# Autodesk Inventor assembly: Хроматографический сортировщик
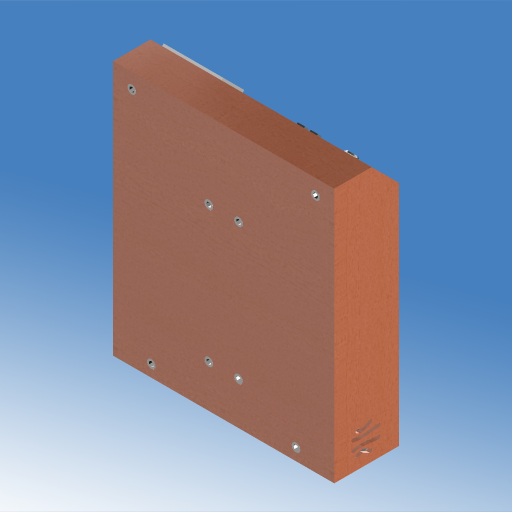
[picture p0: Inventor's stored thumbnail of the model, 512x512]
Saved by Autodesk Inventor 2023 (Build 270158000, 158)
## iProperties
Created: 2022-11-26
Part Number: Хроматографический сортировщик
Document SubType Name: Assembly
Designer: Admin
Author: Admin
## Documents named in this file (32)
- C:\Users\aleks\OneDrive\Рабочий стол\Хроматографический сортировщик\Детали\Хроматографический сортировщик.iam
- C:\Users\aleks\OneDrive\Рабочий стол\Хроматографический сортировщик\Детали\Корпус.ipt
- C:\Users\aleks\OneDrive\Рабочий стол\Хроматографический сортировщик\Детали\Барабан.ipt
- C:\Users\aleks\OneDrive\Рабочий стол\Хроматографический сортировщик\Детали\Короб подшипника.ipt
- C:\Users\aleks\OneDrive\Рабочий стол\Хроматографический сортировщик\Детали\Покупные\Болт М5.ipt
- C:\Users\aleks\OneDrive\Рабочий стол\Хроматографический сортировщик\Детали\Покупные\Гайка М5 стопорная.ipt
- C:\Users\aleks\OneDrive\Рабочий стол\Хроматографический сортировщик\Детали\Покупные\Подшипник.ipt
- C:\Users\aleks\OneDrive\Рабочий стол\Хроматографический сортировщик\Детали\Покупные\Оптический датчик.ipt
- C:\Users\aleks\OneDrive\Рабочий стол\Хроматографический сортировщик\Детали\Покупные\Свая.ipt
- C:\Users\aleks\OneDrive\Рабочий стол\Хроматографический сортировщик\Детали\Покупные\Шаговик\Вал.ipt
- C:\Users\aleks\OneDrive\Рабочий стол\Хроматографический сортировщик\Детали\Покупные\Шаговик\Шаговый мотор.ipt
- C:\Users\aleks\OneDrive\Рабочий стол\Хроматографический сортировщик\Детали\Шевронная маленькая шестерня под мотор.ipt
- C:\Users\aleks\OneDrive\Рабочий стол\Хроматографический сортировщик\Детали\Шевронная планетарная шестерня.ipt
- C:\Users\aleks\OneDrive\Рабочий стол\Хроматографический сортировщик\Детали\Шевронная шестерня для энкодера.ipt
- C:\Users\aleks\OneDrive\Рабочий стол\Хроматографический сортировщик\Детали\Крепёж оптического датчика.ipt
- C:\Users\aleks\OneDrive\Рабочий стол\Хроматографический сортировщик\Детали\Колесо энкодера.ipt
- C:\Users\aleks\OneDrive\Рабочий стол\Хроматографический сортировщик\Детали\Покупные\Болт М3.ipt
- C:\Users\aleks\OneDrive\Рабочий стол\Хроматографический сортировщик\Детали\Покупные\Гайка М3.ipt
- C:\Users\aleks\OneDrive\Рабочий стол\Хроматографический сортировщик\Детали\Покупные\Лазер маленький.ipt
- C:\Users\aleks\OneDrive\Рабочий стол\Хроматографический сортировщик\Детали\Покупные\Лазер.ipt
- C:\Users\aleks\OneDrive\Рабочий стол\Хроматографический сортировщик\Детали\Покупные\Динамик\Динамик.ipt
- C:\Users\aleks\OneDrive\Рабочий стол\Хроматографический сортировщик\Детали\Табличка.ipt
- C:\Users\aleks\OneDrive\Рабочий стол\Хроматографический сортировщик\Детали\Покупные\Кнопки на плате.iam
- C:\Users\aleks\OneDrive\Рабочий стол\Хроматографический сортировщик\Детали\Покупные\Дисплей.ipt
- C:\Users\aleks\OneDrive\Рабочий стол\Хроматографический сортировщик\Детали\Покупные\Кнопка.ipt
- C:\Users\aleks\OneDrive\Рабочий стол\Хроматографический сортировщик\Детали\Колбы\Модель колба коническая 50мл.ipt
- C:\Users\aleks\OneDrive\Рабочий стол\Хроматографический сортировщик\Детали\Покупные\Плата главная.ipt
- C:\Users\aleks\OneDrive\Рабочий стол\Хроматографический сортировщик\Детали\Покупные\Разъём питания.ipt
- C:\Users\aleks\OneDrive\Рабочий стол\Хроматографический сортировщик\Детали\Покупные\Болт М6.ipt
- C:\Users\aleks\OneDrive\Рабочий стол\Хроматографический сортировщик\Детали\Покупные\Гайка М6.ipt
- C:\Users\aleks\OneDrive\Рабочий стол\Хроматографический сортировщик\Детали\Покупные\Болт М4.ipt
- C:\Users\aleks\OneDrive\Рабочий стол\Хроматографический сортировщик\Детали\Покупные\Гайка М4.ipt
## Components (99 placed, 31 different names)
1. Корпус:1 — Совмещение:38, Заподлицо:1, Совмещение:39, Совмещение:40, Заподлицо:2, Совмещение:41, Совмещение:42, Совмещение:43, Совмещение:44, Совмещение:51, Совмещение:52, Совмещение:53, Угол:3, Угол:4, Совмещение:72, Совмещение:73, Совмещение:74, Заподлицо:6, Совмещение:75, Совмещение:76, Совмещение:77, Совмещение:78, Совмещение:80, Угол:5, Совмещение:81, Угол:6, Совмещение:82, Совмещение:85, Совмещение:86, Совмещение:87, Совмещение:88, Совмещение:89, Совмещение:91, Совмещение:92, Совмещение:93, Совмещение:94, Совмещение:96, Совмещение:97, Совмещение:98, Совмещение:101, Совмещение:102, Совмещение:103, Совмещение:104, Совмещение:128, Совмещение:129, Совмещение:130, Совмещение:131, Совмещение:132, Совмещение:133, Совмещение:134, Совмещение:137, Совмещение:138, Совмещение:139, Совмещение:140, Совмещение:141, Совмещение:142, Заподлицо:17, Заподлицо:18, Заподлицо:19, Заподлицо:20, Заподлицо:21, Заподлицо:22, Заподлицо:23, Заподлицо:24, Угол:7, Угол:8, Угол:9, Угол:10, Совмещение:148, Угол:11, Заподлицо:27, Угол:12, Угол:13, Заподлицо:28, Совмещение:156, Совмещение:157, Совмещение:158, Совмещение:159, Угол:15, Угол:16, Угол:17, Угол:18, Заподлицо:29, Заподлицо:30, Заподлицо:31, Заподлицо:32, Совмещение:164, Совмещение:165, Совмещение:166, Совмещение:167, Совмещение:168, Совмещение:169, Совмещение:170, Совмещение:171, Совмещение:172, Угол:19, Угол:20, Угол:21, Угол:22, Заподлицо:36, Заподлицо:37, Заподлицо:38, Заподлицо:39, Заподлицо:40, Заподлицо:41, Заподлицо:42, Заподлицо:43, Угол:23, Угол:24, Угол:25, Угол:26
2. Барабан:1 — Совмещение:25, Совмещение:27, Совмещение:28, Совмещение:29, Совмещение:30, Совмещение:31, Совмещение:32, Совмещение:33, Совмещение:34, Совмещение:35, Совмещение:36, Совмещение:37, Совмещение:38, Заподлицо:1, Совмещение:49, ЗубчПер:5, Совмещение:108, Совмещение:109, Совмещение:110, Совмещение:111, Совмещение:112, Совмещение:113, Совмещение:114, Совмещение:115, Совмещение:116, Совмещение:117, Совмещение:118, Совмещение:119, Совмещение:120, Совмещение:121, Совмещение:122, Совмещение:123
3. Короб подшипника:1 — Совмещение:3, Совмещение:13, Совмещение:17, Совмещение:18, Совмещение:25, Совмещение:27, Совмещение:28
4. Короб подшипника:2 — Совмещение:4, Совмещение:10, Совмещение:16, Совмещение:23, Совмещение:24, Совмещение:29, Совмещение:30, Совмещение:31
5. Короб подшипника:3 — Совмещение:1, Совмещение:15, Совмещение:21, Совмещение:22, Совмещение:32, Совмещение:33, Совмещение:34
6. Короб подшипника:4 — Совмещение:2, Совмещение:14, Совмещение:19, Совмещение:20, Совмещение:35, Совмещение:36, Совмещение:37
7. Болт М5:1 — Совмещение:11, Совмещение:20
8. Гайка М5 стопорная:1 — Совмещение:8, Совмещение:19
9. Подшипник:1 — Совмещение:2, Совмещение:8, Совмещение:11, Совмещение:14
10. Болт М5:2 — Совмещение:12, Совмещение:22
11. Гайка М5 стопорная:2 — Совмещение:7, Совмещение:12, Совмещение:21
12. Подшипник:2 — Совмещение:1, Совмещение:7, Совмещение:15
13. Болт М5:3 — Совмещение:10, Совмещение:24
14. Гайка М5 стопорная:3 — Совмещение:6, Совмещение:23
15. Подшипник:3 — Совмещение:4, Совмещение:6, Совмещение:16
16. Болт М5:4 — Совмещение:9, Совмещение:18
17. Гайка М5 стопорная:4 — Совмещение:5, Совмещение:17
18. Подшипник:4 — Совмещение:3, Совмещение:5, Совмещение:9, Совмещение:13
19. Оптический датчик:1 — Совмещение:54, Совмещение:55, Совмещение:56, Совмещение:58, Совмещение:63, Совмещение:64
20. Подшипник:5 — Совмещение:40, Заподлицо:2
21. Свая:1 — Совмещение:39, Совмещение:41, Совмещение:50, Заподлицо:4, Совмещение:57, ЗубчПер:4
22. Вал:1 — Совмещение:45, Совмещение:46, Совмещение:154, Совмещение:155, Угол:14
23. Шаговый мотор:1 — Совмещение:42, Совмещение:43, Совмещение:44, Совмещение:45, Совмещение:46, Совмещение:149, Совмещение:150, Совмещение:151
24. Шевронная маленькая шестерня под мотор:1 — Заподлицо:3, ЗубчПер:1, ЗубчПер:2, Совмещение:154, Совмещение:155, Угол:14
25. Шевронная планетарная шестерня:1 — Совмещение:49, Заподлицо:3, ЗубчПер:2, ЗубчПер:5
26. Шевронная шестерня для энкодера:1 — Совмещение:50, Заподлицо:4, ЗубчПер:1, ЗубчПер:3, ЗубчПер:4
27. Крепёж оптического датчика:1 — Совмещение:51, Совмещение:52, Совмещение:53, Совмещение:54, Совмещение:55, Совмещение:56, Совмещение:59, Совмещение:60, Совмещение:61, Совмещение:62, Совмещение:65, Совмещение:68, Угол:1, Совмещение:69, Угол:2
28. Колесо энкодера:1 — Совмещение:57, Совмещение:58, ЗубчПер:3
29. Болт М3:1 — Совмещение:59, Заподлицо:5, Совмещение:71
30. Болт М3:2 — Совмещение:60, Заподлицо:5, Совмещение:65, Совмещение:70
31. Болт М3:3 — Совмещение:61, Совмещение:63, Совмещение:66, ЗубчПер:6
32. Болт М3:4 — Совмещение:62, Совмещение:64, Совмещение:67, ЗубчПер:7
33. Гайка М3:1 — Совмещение:71, Угол:4, Совмещение:72
34. Гайка М3:2 — Совмещение:70, Угол:3, Совмещение:73
35. Гайка М3:3 — Совмещение:66, Совмещение:68, Угол:1, ЗубчПер:6
36. Гайка М3:4 — Совмещение:67, Совмещение:69, Угол:2, ЗубчПер:7
37. Лазер маленький:1 — Совмещение:75, Совмещение:77
38. Лазер маленький:2 — Совмещение:76, Совмещение:78
39. Лазер:1 — Совмещение:74, Заподлицо:6
40. Болт М3:5 — Совмещение:84, Совмещение:85
41. Болт М3:6 — Совмещение:83, Совмещение:86
42. Гайка М3:5 — Совмещение:80, Угол:5, Заподлицо:7, Совмещение:83
43. Гайка М3:6 — Совмещение:81, Угол:6, Заподлицо:7, Совмещение:82, Совмещение:84
44. Динамик:1 — Совмещение:87, Совмещение:90
45. Динамик:2 — Совмещение:88, Совмещение:89, Совмещение:90
46. Табличка:1 — Совмещение:91, Совмещение:92, Совмещение:93
47. Кнопки на плате:1 [sub-assembly] — Совмещение:97, Совмещение:98, Совмещение:104
48. Дисплей:1 — Совмещение:96, Совмещение:102, Совмещение:103
49. Кнопка:1 — Совмещение:94, Совмещение:101
50. Модель колба коническая 50мл:1 — Совмещение:114, Совмещение:122
51. Модель колба коническая 50мл:2 — Совмещение:115, Совмещение:121
52. Модель колба коническая 50мл:3 — Совмещение:110, Совмещение:118
53. Модель колба коническая 50мл:4 — Совмещение:113, Совмещение:123
54. Модель колба коническая 50мл:5 — Совмещение:112, Совмещение:116
55. Модель колба коническая 50мл:6 — Совмещение:111, Совмещение:117
56. Модель колба коническая 50мл:7 — Совмещение:109, Совмещение:119
57. Модель колба коническая 50мл:8 — Совмещение:108, Совмещение:120
58. Плата главная:1 — Совмещение:124, Совмещение:125, Совмещение:126, Совмещение:127, Совмещение:129, Совмещение:135, Совмещение:136
59. Болт М3:7 — Заподлицо:8, Совмещение:124, Заподлицо:16, Совмещение:179
60. Болт М3:8 — Заподлицо:9, Заподлицо:10, Совмещение:126, Заподлицо:14, Заподлицо:15, Совмещение:177
61. Болт М3:9 — Заподлицо:10, Совмещение:125, Заподлицо:14, Совмещение:178
62. Болт М3:10 — Заподлицо:8, Заподлицо:9, Совмещение:127, Совмещение:128, Заподлицо:15, Заподлицо:16, Совмещение:136, Совмещение:180
63. Гайка М3:7 — Совмещение:133, Совмещение:134, Заподлицо:11
64. Гайка М3:8 — Совмещение:131, Заподлицо:12, Совмещение:135
65. Гайка М3:9 — Совмещение:132, Заподлицо:11, Заподлицо:12, Заподлицо:13
66. Гайка М3:10 — Совмещение:130, Заподлицо:13
67. Разъём питания:1 — Совмещение:137, Совмещение:138
68. Болт М6:1 — Совмещение:141, Заподлицо:17, Совмещение:147
69. Болт М6:2 — Совмещение:140, Заподлицо:20, Совмещение:146
70. Болт М6:3 — Совмещение:142, Заподлицо:18, Совмещение:144
71. Болт М6:4 — Совмещение:139, Заподлицо:19, Совмещение:143
72. Гайка М6:1 — Совмещение:144, Заподлицо:24, Угол:7
73. Гайка М6:2 — Совмещение:143, Заподлицо:23, Угол:8
74. Гайка М6:3 — Совмещение:146, Заподлицо:21, Угол:10
75. Гайка М6:4 — Совмещение:147, Заподлицо:22, Угол:9
76. Болт М4:1 — Совмещение:149, Заподлицо:26, Совмещение:153
77. Гайка М4:1 — Совмещение:152, Угол:13, Заподлицо:28
78. Болт М4:2 — Совмещение:150, Заподлицо:26, Совмещение:151, Совмещение:152
79. Гайка М4:2 — Совмещение:153, Заподлицо:27, Угол:12
80. Болт М3:11 — Совмещение:158, Совмещение:161, Заподлицо:34
81. Гайка М3:11 — Совмещение:162, Угол:16, Заподлицо:29
82. Болт М3:12 — Совмещение:156, Совмещение:162, Заподлицо:34, Заподлицо:35
83. Гайка М3:12 — Совмещение:160, Угол:15, Заподлицо:30
84. Болт М3:13 — Совмещение:157, Совмещение:160, Заподлицо:33, Заподлицо:35, Совмещение:164
85. Гайка М3:13 — Совмещение:161, Угол:17, Заподлицо:31
86. Болт М3:14 — Совмещение:159, Совмещение:163, Заподлицо:33
87. Гайка М3:14 — Совмещение:163, Угол:18, Заподлицо:32
88. Болт М6:5 — Совмещение:168, Совмещение:176, Заподлицо:38
89. Гайка М6:5 — Совмещение:169, Угол:21, Совмещение:176
90. Болт М6:6 — Совмещение:166, Совмещение:173, Заподлицо:37
91. Гайка М6:6 — Совмещение:170, Угол:22, Совмещение:175
92. Болт М6:7 — Совмещение:165, Совмещение:174, Заподлицо:36
93. Гайка М6:7 — Совмещение:172, Угол:19, Совмещение:173
94. Болт М6:8 — Совмещение:167, Совмещение:175, Заподлицо:39
95. Гайка М6:8 — Совмещение:171, Угол:20, Совмещение:174
96. Гайка М3:15 — Совмещение:177, Заподлицо:41, Угол:25
97. Гайка М3:16 — Совмещение:178, Заподлицо:42, Угол:24
98. Гайка М3:17 — Совмещение:179, Заподлицо:43, Угол:23
99. Гайка М3:18 — Совмещение:180, Заподлицо:40, Угол:26
## Relationships (245: Mate 169, Flush 43, Angle 26, RelateRotation 7)
- Совмещение:1 [Mate]: Короб подшипника:3 ↔ Подшипник:2
- Совмещение:2 [Mate]: Короб подшипника:4 ↔ Подшипник:1
- Совмещение:3 [Mate]: Короб подшипника:1 ↔ Подшипник:4
- Совмещение:4 [Mate]: Короб подшипника:2 ↔ Подшипник:3
- Совмещение:5 [Mate]: Гайка М5 стопорная:4 ↔ Подшипник:4
- Совмещение:6 [Mate]: Гайка М5 стопорная:3 ↔ Подшипник:3
- Совмещение:7 [Mate]: Гайка М5 стопорная:2 ↔ Подшипник:2
- Совмещение:8 [Mate]: Гайка М5 стопорная:1 ↔ Подшипник:1
- Совмещение:9 [Mate]: Болт М5:4 ↔ Подшипник:4
- Совмещение:10 [Mate]: Короб подшипника:2 ↔ Болт М5:3
- Совмещение:11 [Mate]: Болт М5:1 ↔ Подшипник:1
- Совмещение:12 [Mate]: Болт М5:2 ↔ Гайка М5 стопорная:2
- Совмещение:13 [Mate] (0.5 mm): Короб подшипника:1 ↔ Подшипник:4
- Совмещение:14 [Mate] (0.5 mm): Короб подшипника:4 ↔ Подшипник:1
- Совмещение:15 [Mate] (0.5 mm): Короб подшипника:3 ↔ Подшипник:2
- Совмещение:16 [Mate] (0.5 mm): Короб подшипника:2 ↔ Подшипник:3
- Совмещение:17 [Mate]: Короб подшипника:1 ↔ Гайка М5 стопорная:4
- Совмещение:18 [Mate]: Короб подшипника:1 ↔ Болт М5:4
- Совмещение:19 [Mate]: Короб подшипника:4 ↔ Гайка М5 стопорная:1
- Совмещение:20 [Mate]: Короб подшипника:4 ↔ Болт М5:1
- Совмещение:21 [Mate]: Короб подшипника:3 ↔ Гайка М5 стопорная:2
- Совмещение:22 [Mate]: Короб подшипника:3 ↔ Болт М5:2
- Совмещение:23 [Mate]: Короб подшипника:2 ↔ Гайка М5 стопорная:3
- Совмещение:24 [Mate]: Короб подшипника:2 ↔ Болт М5:3
- Совмещение:25 [Mate] (0.1 mm): Барабан:1 ↔ Короб подшипника:1
- Совмещение:27 [Mate]: Барабан:1 ↔ Короб подшипника:1
- Совмещение:28 [Mate] (0.1 mm): Барабан:1 ↔ Короб подшипника:1
- Совмещение:29 [Mate] (0.1 mm): Барабан:1 ↔ Короб подшипника:2
- Совмещение:30 [Mate] (0.1 mm): Барабан:1 ↔ Короб подшипника:2
- Совмещение:31 [Mate]: Барабан:1 ↔ Короб подшипника:2
- Совмещение:32 [Mate] (0.1 mm): Барабан:1 ↔ Короб подшипника:3
- Совмещение:33 [Mate] (0.1 mm): Барабан:1 ↔ Короб подшипника:3
- Совмещение:34 [Mate]: Барабан:1 ↔ Короб подшипника:3
- Совмещение:35 [Mate]: Барабан:1 ↔ Короб подшипника:4
- Совмещение:36 [Mate] (0.1 mm): Барабан:1 ↔ Короб подшипника:4
- Совмещение:37 [Mate] (0.1 mm): Барабан:1 ↔ Короб подшипника:4
- Совмещение:38 [Mate]: Корпус:1 ↔ Барабан:1
- Заподлицо:1 [Flush] (-62.5 mm): Корпус:1 ↔ Барабан:1
- Совмещение:39 [Mate]: Корпус:1 ↔ Свая:1
- Совмещение:40 [Mate]: Корпус:1 ↔ Подшипник:5
- Заподлицо:2 [Flush]: Корпус:1 ↔ Подшипник:5
- Совмещение:41 [Mate]: Корпус:1 ↔ Свая:1
- Совмещение:42 [Mate]: Корпус:1 ↔ Шаговый мотор:1
- Совмещение:43 [Mate]: Корпус:1 ↔ Шаговый мотор:1
- Совмещение:44 [Mate]: Корпус:1 ↔ Шаговый мотор:1
- Совмещение:45 [Mate]: Вал:1 ↔ Шаговый мотор:1
- Совмещение:46 [Mate]: Вал:1 ↔ Шаговый мотор:1
- Совмещение:49 [Mate]: Барабан:1 ↔ Шевронная планетарная шестерня:1
- Заподлицо:3 [Flush]: Шевронная маленькая шестерня под мотор:1 ↔ Шевронная планетарная шестерня:1
- Совмещение:50 [Mate]: Свая:1 ↔ Шевронная шестерня для энкодера:1
- Заподлицо:4 [Flush]: Свая:1 ↔ Шевронная шестерня для энкодера:1
- ЗубчПер:1 [RelateRotation] (1 ul): Шевронная маленькая шестерня под мотор:1 ↔ Шевронная шестерня для энкодера:1
- ЗубчПер:2 [RelateRotation] (0.375 ul): Шевронная маленькая шестерня под мотор:1 ↔ Шевронная планетарная шестерня:1
- Совмещение:51 [Mate]: Корпус:1 ↔ Крепёж оптического датчика:1
- Совмещение:52 [Mate]: Корпус:1 ↔ Крепёж оптического датчика:1
- Совмещение:53 [Mate]: Корпус:1 ↔ Крепёж оптического датчика:1
- Совмещение:54 [Mate]: Оптический датчик:1 ↔ Крепёж оптического датчика:1
- Совмещение:55 [Mate]: Оптический датчик:1 ↔ Крепёж оптического датчика:1
- Совмещение:56 [Mate]: Оптический датчик:1 ↔ Крепёж оптического датчика:1
- Совмещение:57 [Mate]: Свая:1 ↔ Колесо энкодера:1
- Совмещение:58 [Mate]: Оптический датчик:1 ↔ Колесо энкодера:1
- ЗубчПер:3 [RelateRotation] (1 ul): Шевронная шестерня для энкодера:1 ↔ Колесо энкодера:1
- ЗубчПер:4 [RelateRotation] (1 ul): Свая:1 ↔ Шевронная шестерня для энкодера:1
- ЗубчПер:5 [RelateRotation] (1 ul): Барабан:1 ↔ Шевронная планетарная шестерня:1
- Совмещение:59 [Mate]: Крепёж оптического датчика:1 ↔ Болт М3:1
- Совмещение:60 [Mate]: Крепёж оптического датчика:1 ↔ Болт М3:2
- Совмещение:61 [Mate]: Крепёж оптического датчика:1 ↔ Болт М3:3
- Совмещение:62 [Mate]: Крепёж оптического датчика:1 ↔ Болт М3:4
- Совмещение:63 [Mate]: Оптический датчик:1 ↔ Болт М3:3
- Совмещение:64 [Mate]: Оптический датчик:1 ↔ Болт М3:4
- Заподлицо:5 [Flush]: Болт М3:1 ↔ Болт М3:2
- Совмещение:65 [Mate]: Крепёж оптического датчика:1 ↔ Болт М3:2
- Совмещение:66 [Mate]: Болт М3:3 ↔ Гайка М3:3
- Совмещение:67 [Mate]: Болт М3:4 ↔ Гайка М3:4
- Совмещение:68 [Mate]: Крепёж оптического датчика:1 ↔ Гайка М3:3
- Угол:1 [Angle] (0 deg): Крепёж оптического датчика:1 ↔ Гайка М3:3
- Совмещение:69 [Mate]: Крепёж оптического датчика:1 ↔ Гайка М3:4
- Угол:2 [Angle] (0 deg): Крепёж оптического датчика:1 ↔ Гайка М3:4
- ЗубчПер:6 [RelateRotation] (1 ul): Болт М3:3 ↔ Гайка М3:3
- ЗубчПер:7 [RelateRotation] (1 ul): Болт М3:4 ↔ Гайка М3:4
- Совмещение:70 [Mate]: Болт М3:2 ↔ Гайка М3:2
- Совмещение:71 [Mate]: Болт М3:1 ↔ Гайка М3:1
- Угол:3 [Angle] (0 deg): Корпус:1 ↔ Гайка М3:2
- Угол:4 [Angle] (0 deg): Корпус:1 ↔ Гайка М3:1
- Совмещение:72 [Mate]: Корпус:1 ↔ Гайка М3:1
- Совмещение:73 [Mate]: Корпус:1 ↔ Гайка М3:2
- Совмещение:74 [Mate]: Корпус:1 ↔ Лазер:1
- Заподлицо:6 [Flush]: Корпус:1 ↔ Лазер:1
- Совмещение:75 [Mate]: Корпус:1 ↔ Лазер маленький:1
- Совмещение:76 [Mate]: Корпус:1 ↔ Лазер маленький:2
- Совмещение:77 [Mate]: Корпус:1 ↔ Лазер маленький:1
- Совмещение:78 [Mate]: Корпус:1 ↔ Лазер маленький:2
- Совмещение:80 [Mate]: Корпус:1 ↔ Гайка М3:5
- Угол:5 [Angle] (0 deg): Корпус:1 ↔ Гайка М3:5
- Совмещение:81 [Mate]: Корпус:1 ↔ Гайка М3:6
- Угол:6 [Angle] (0 deg): Корпус:1 ↔ Гайка М3:6
- Заподлицо:7 [Flush]: Гайка М3:5 ↔ Гайка М3:6
- Совмещение:82 [Mate]: Корпус:1 ↔ Гайка М3:6
- Совмещение:83 [Mate]: Болт М3:6 ↔ Гайка М3:5
- Совмещение:84 [Mate]: Болт М3:5 ↔ Гайка М3:6
- Совмещение:85 [Mate]: Корпус:1 ↔ Болт М3:5
- Совмещение:86 [Mate]: Корпус:1 ↔ Болт М3:6
- Совмещение:87 [Mate]: Корпус:1 ↔ Динамик:1
- Совмещение:88 [Mate]: Корпус:1 ↔ Динамик:2
- Совмещение:89 [Mate]: Корпус:1 ↔ Динамик:2
- Совмещение:90 [Mate]: Динамик:1 ↔ Динамик:2
- Совмещение:91 [Mate]: Корпус:1 ↔ Табличка:1
- Совмещение:92 [Mate]: Корпус:1 ↔ Табличка:1
- Совмещение:93 [Mate]: Корпус:1 ↔ Табличка:1
- Совмещение:94 [Mate]: Корпус:1 ↔ Кнопка:1
- Совмещение:96 [Mate]: Корпус:1 ↔ Дисплей:1
- Совмещение:97 [Mate]: Корпус:1 ↔ Кнопки на плате:1
- Совмещение:98 [Mate]: Корпус:1 ↔ Кнопки на плате:1
- Совмещение:101 [Mate]: Корпус:1 ↔ Кнопка:1
- Совмещение:102 [Mate]: Корпус:1 ↔ Дисплей:1
- Совмещение:103 [Mate]: Корпус:1 ↔ Дисплей:1
- Совмещение:104 [Mate]: Корпус:1 ↔ Кнопки на плате:1
- Совмещение:108 [Mate]: Барабан:1 ↔ Модель колба коническая 50мл:8
- Совмещение:109 [Mate]: Барабан:1 ↔ Модель колба коническая 50мл:7
- Совмещение:110 [Mate]: Барабан:1 ↔ Модель колба коническая 50мл:3
- Совмещение:111 [Mate]: Барабан:1 ↔ Модель колба коническая 50мл:6
- Совмещение:112 [Mate]: Барабан:1 ↔ Модель колба коническая 50мл:5
- Совмещение:113 [Mate]: Барабан:1 ↔ Модель колба коническая 50мл:4
- Совмещение:114 [Mate]: Барабан:1 ↔ Модель колба коническая 50мл:1
- Совмещение:115 [Mate]: Барабан:1 ↔ Модель колба коническая 50мл:2
- Совмещение:116 [Mate]: Барабан:1 ↔ Модель колба коническая 50мл:5
- Совмещение:117 [Mate]: Барабан:1 ↔ Модель колба коническая 50мл:6
- Совмещение:118 [Mate]: Барабан:1 ↔ Модель колба коническая 50мл:3
- Совмещение:119 [Mate]: Барабан:1 ↔ Модель колба коническая 50мл:7
- Совмещение:120 [Mate]: Барабан:1 ↔ Модель колба коническая 50мл:8
- Совмещение:121 [Mate]: Барабан:1 ↔ Модель колба коническая 50мл:2
- Совмещение:122 [Mate]: Барабан:1 ↔ Модель колба коническая 50мл:1
- Совмещение:123 [Mate]: Барабан:1 ↔ Модель колба коническая 50мл:4
- Заподлицо:8 [Flush]: Болт М3:7 ↔ Болт М3:10
- Заподлицо:9 [Flush]: Болт М3:8 ↔ Болт М3:10
- Заподлицо:10 [Flush]: Болт М3:8 ↔ Болт М3:9
- Совмещение:124 [Mate]: Плата главная:1 ↔ Болт М3:7
- Совмещение:125 [Mate]: Плата главная:1 ↔ Болт М3:9
- Совмещение:126 [Mate]: Плата главная:1 ↔ Болт М3:8
- Совмещение:127 [Mate]: Плата главная:1 ↔ Болт М3:10
- Совмещение:128 [Mate]: Корпус:1 ↔ Болт М3:10
- Совмещение:129 [Mate]: Корпус:1 ↔ Плата главная:1
- Совмещение:130 [Mate]: Корпус:1 ↔ Гайка М3:10
- Совмещение:131 [Mate]: Корпус:1 ↔ Гайка М3:8
- Совмещение:132 [Mate]: Корпус:1 ↔ Гайка М3:9
- Совмещение:133 [Mate]: Корпус:1 ↔ Гайка М3:7
- Совмещение:134 [Mate]: Корпус:1 ↔ Гайка М3:7
- Заподлицо:11 [Flush]: Гайка М3:7 ↔ Гайка М3:9
- Заподлицо:12 [Flush]: Гайка М3:8 ↔ Гайка М3:9
- Заподлицо:13 [Flush]: Гайка М3:9 ↔ Гайка М3:10
- Совмещение:135 [Mate]: Плата главная:1 ↔ Гайка М3:8
- Заподлицо:14 [Flush]: Болт М3:8 ↔ Болт М3:9
- Заподлицо:15 [Flush]: Болт М3:8 ↔ Болт М3:10
- Заподлицо:16 [Flush]: Болт М3:7 ↔ Болт М3:10
- Совмещение:136 [Mate]: Плата главная:1 ↔ Болт М3:10
- Совмещение:137 [Mate]: Корпус:1 ↔ Разъём питания:1
- Совмещение:138 [Mate]: Корпус:1 ↔ Разъём питания:1
- Совмещение:139 [Mate]: Корпус:1 ↔ Болт М6:4
- Совмещение:140 [Mate]: Корпус:1 ↔ Болт М6:2
- Совмещение:141 [Mate]: Корпус:1 ↔ Болт М6:1
- Совмещение:142 [Mate]: Корпус:1 ↔ Болт М6:3
- Заподлицо:17 [Flush]: Корпус:1 ↔ Болт М6:1
- Заподлицо:18 [Flush]: Корпус:1 ↔ Болт М6:3
- Заподлицо:19 [Flush]: Корпус:1 ↔ Болт М6:4
- Заподлицо:20 [Flush]: Корпус:1 ↔ Болт М6:2
- Совмещение:143 [Mate]: Болт М6:4 ↔ Гайка М6:2
- Совмещение:144 [Mate]: Болт М6:3 ↔ Гайка М6:1
- Совмещение:146 [Mate]: Болт М6:2 ↔ Гайка М6:3
- Совмещение:147 [Mate]: Болт М6:1 ↔ Гайка М6:4
- Заподлицо:21 [Flush]: Корпус:1 ↔ Гайка М6:3
- Заподлицо:22 [Flush]: Корпус:1 ↔ Гайка М6:4
- Заподлицо:23 [Flush]: Корпус:1 ↔ Гайка М6:2
- Заподлицо:24 [Flush]: Корпус:1 ↔ Гайка М6:1
- Угол:7 [Angle] (0 deg): Корпус:1 ↔ Гайка М6:1
- Угол:8 [Angle] (0 deg): Корпус:1 ↔ Гайка М6:2
- Угол:9 [Angle] (0 deg): Корпус:1 ↔ Гайка М6:4
- Угол:10 [Angle] (0 deg): Корпус:1 ↔ Гайка М6:3
- Совмещение:148 [Mate]: Корпус:1
- Угол:11 [Angle] (15 deg): Корпус:1
- Заподлицо:25 [Flush] (80 mm)
- Совмещение:149 [Mate]: Шаговый мотор:1 ↔ Болт М4:1
- Совмещение:150 [Mate]: Шаговый мотор:1 ↔ Болт М4:2
- Заподлицо:26 [Flush]: Болт М4:1 ↔ Болт М4:2
- Совмещение:151 [Mate]: Шаговый мотор:1 ↔ Болт М4:2
- Совмещение:152 [Mate]: Гайка М4:1 ↔ Болт М4:2
- Совмещение:153 [Mate]: Болт М4:1 ↔ Гайка М4:2
- Заподлицо:27 [Flush]: Корпус:1 ↔ Гайка М4:2
- Угол:12 [Angle] (0 deg): Корпус:1 ↔ Гайка М4:2
- Угол:13 [Angle] (0 deg): Корпус:1 ↔ Гайка М4:1
- Заподлицо:28 [Flush]: Корпус:1 ↔ Гайка М4:1
- Совмещение:154 [Mate]: Вал:1 ↔ Шевронная маленькая шестерня под мотор:1
- Совмещение:155 [Mate] (2 mm): Вал:1 ↔ Шевронная маленькая шестерня под мотор:1
- Угол:14 [Angle] (0 deg): Вал:1 ↔ Шевронная маленькая шестерня под мотор:1
- Совмещение:156 [Mate]: Корпус:1 ↔ Болт М3:12
- Совмещение:157 [Mate]: Корпус:1 ↔ Болт М3:13
- Совмещение:158 [Mate]: Корпус:1 ↔ Болт М3:11
- Совмещение:159 [Mate]: Корпус:1 ↔ Болт М3:14
- Совмещение:160 [Mate]: Гайка М3:12 ↔ Болт М3:13
- Совмещение:161 [Mate]: Болт М3:11 ↔ Гайка М3:13
- Совмещение:162 [Mate]: Гайка М3:11 ↔ Болт М3:12
- Совмещение:163 [Mate]: Болт М3:14 ↔ Гайка М3:14
- Угол:15 [Angle] (0 deg): Корпус:1 ↔ Гайка М3:12
- Угол:16 [Angle] (0 deg): Корпус:1 ↔ Гайка М3:11
- Угол:17 [Angle] (0 deg): Корпус:1 ↔ Гайка М3:13
- Угол:18 [Angle] (0 deg): Корпус:1 ↔ Гайка М3:14
- Заподлицо:29 [Flush]: Корпус:1 ↔ Гайка М3:11
- Заподлицо:30 [Flush]: Корпус:1 ↔ Гайка М3:12
- Заподлицо:31 [Flush]: Корпус:1 ↔ Гайка М3:13
- Заподлицо:32 [Flush]: Корпус:1 ↔ Гайка М3:14
- Заподлицо:33 [Flush]: Болт М3:13 ↔ Болт М3:14
- Заподлицо:34 [Flush]: Болт М3:11 ↔ Болт М3:12
- Заподлицо:35 [Flush]: Болт М3:12 ↔ Болт М3:13
- Совмещение:164 [Mate] (2 mm): Корпус:1 ↔ Болт М3:13
- Совмещение:165 [Mate]: Корпус:1 ↔ Болт М6:7
- Совмещение:166 [Mate]: Корпус:1 ↔ Болт М6:6
- Совмещение:167 [Mate]: Корпус:1 ↔ Болт М6:8
- Совмещение:168 [Mate]: Корпус:1 ↔ Болт М6:5
- Совмещение:169 [Mate]: Корпус:1 ↔ Гайка М6:5
- Совмещение:170 [Mate]: Корпус:1 ↔ Гайка М6:6
- Совмещение:171 [Mate]: Корпус:1 ↔ Гайка М6:8
- Совмещение:172 [Mate]: Корпус:1 ↔ Гайка М6:7
- Угол:19 [Angle] (0 deg): Корпус:1 ↔ Гайка М6:7
- Угол:20 [Angle] (0 deg): Корпус:1 ↔ Гайка М6:8
- Угол:21 [Angle] (0 deg): Корпус:1 ↔ Гайка М6:5
- Угол:22 [Angle] (0 deg): Корпус:1 ↔ Гайка М6:6
- Совмещение:173 [Mate]: Болт М6:6 ↔ Гайка М6:7
- Совмещение:174 [Mate]: Болт М6:7 ↔ Гайка М6:8
- Совмещение:175 [Mate]: Гайка М6:6 ↔ Болт М6:8
- Совмещение:176 [Mate]: Болт М6:5 ↔ Гайка М6:5
- Заподлицо:36 [Flush]: Корпус:1 ↔ Болт М6:7
- Заподлицо:37 [Flush]: Корпус:1 ↔ Болт М6:6
- Заподлицо:38 [Flush]: Корпус:1 ↔ Болт М6:5
- Заподлицо:39 [Flush]: Корпус:1 ↔ Болт М6:8
- Совмещение:177 [Mate]: Болт М3:8 ↔ Гайка М3:15
- Совмещение:178 [Mate]: Болт М3:9 ↔ Гайка М3:16
- Совмещение:179 [Mate]: Болт М3:7 ↔ Гайка М3:17
- Совмещение:180 [Mate]: Болт М3:10 ↔ Гайка М3:18
- Заподлицо:40 [Flush]: Корпус:1 ↔ Гайка М3:18
- Заподлицо:41 [Flush]: Корпус:1 ↔ Гайка М3:15
- Заподлицо:42 [Flush]: Корпус:1 ↔ Гайка М3:16
- Заподлицо:43 [Flush]: Корпус:1 ↔ Гайка М3:17
- Угол:23 [Angle] (0 deg): Корпус:1 ↔ Гайка М3:17
- Угол:24 [Angle] (0 deg): Корпус:1 ↔ Гайка М3:16
- Угол:25 [Angle] (0 deg): Корпус:1 ↔ Гайка М3:15
- Угол:26 [Angle] (0 deg): Корпус:1 ↔ Гайка М3:18
